# Autodesk Inventor assembly: Spring Assembly
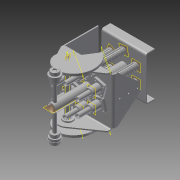
[picture p0: Inventor's stored thumbnail of the model, 180x180]
Saved by Autodesk Inventor 2014 (Build 180170000, 170)
## iProperties
Created: 2014-01-12
Part Number: Spring Assembly
Document SubType Name: Assembly
Designer: Andrew Toennies
Mass: 3782.05 g
Surface Area: 3929.11 cm^2
Volume: 481.789 cm^3
Density: 7.85 g/cm^3
Author: Andrew Toennies
## Documents named in this file (12)
- C:\Users\Andrew Toennies\Documents\GitHub\2014buildCAD\Shooter\Launching Mechanism\Spring Assembly.iam
- C:\Users\Andrew Toennies\Documents\GitHub\2014buildCAD\Shooter\Launching Mechanism\Plate (Front).ipt
- C:\Users\Andrew Toennies\Documents\GitHub\2014buildCAD\Shooter\Launching Mechanism\Spring 9657K213.ipt
- C:\Users\Andrew Toennies\Documents\GitHub\2014buildCAD\Shooter\Launching Mechanism\Shaft (0.500 Aluminum.ipt
- C:\Users\Andrew Toennies\Documents\GitHub\2014buildCAD\Shooter\Launching Mechanism\Plate 2 (Back).ipt
- C:\Users\Andrew Toennies\Documents\GitHub\2014buildCAD\Shooter\Launching Mechanism\Linear Bearing 6483K630.ipt
- C:\Users\Andrew Toennies\Documents\GitHub\2014buildCAD\Shooter\Launching Mechanism\Nautilus Cam.ipt
- C:\Users\Andrew Toennies\Documents\GitHub\2014buildCAD\Shooter\Launching Mechanism\Steel Pipe.ipt
- C:\Users\Andrew Toennies\Documents\GitHub\2014buildCAD\Shooter\Launching Mechanism\Steel Shaft.ipt
- C:\Users\Andrew Toennies\Documents\GitHub\2014buildCAD\Shooter\Launching Mechanism\Steel Shaft 2.ipt
- C:\Users\Andrew Toennies\Documents\GitHub\2014buildCAD\Shooter\Bearing ID 0.500 Hex OD 1.125.ipt
- C:\Users\Andrew Toennies\Documents\GitHub\2014buildCAD\Shooter\Bearing .5 Shaft 6384K610.ipt
## Components (29 placed, 11 different names)
1. Plate (Front):1 — Flush:1, Flush:2, Flush:3, Flush:4, Flush:5, Flush:6, Flush:7, Mate:7, Mate:8, Flush:8, Mate:9, Flush:9, Mate:10, Flush:10, Mate:11, Flush:11, Mate:12, Flush:12, Mate:37, Mate:55, Flush:19
2. Plate 2 (Back):1 — Mate:13, Mate:14, Mate:16, Mate:17, Mate:18, Mate:19, Mate:20, Mate:21, Mate:22, Mate:23, Mate:24, Mate:25, Mate:26, Mate:27, Mate:28, Mate:29, Mate:30, Mate:31, Mate:32, Mate:33, Mate:34, Mate:48, Mate:49, Mate:50, Mate:51, Mate:52, Mate:53, Mate:55
3. Nautilus Cam:1 — Flush:13, Flush:14, Flush:17, Mate:48, Flush:18, Tangent:1
4. Nautilus Cam:2 — Flush:13, Flush:14, Mate:41, Mate:42, Mate:49, Flush:20
5. Steel Pipe:1 — Mate:37, Mate:44, Mate:66, Flush:19
6. Steel Shaft:1 — Mate:41, Mate:42, Flush:17, Mate:54
7. Steel Shaft 2:1 — Mate:44, Mate:64, Mate:65, Mate:66
8. Bearing ID 0.500 Hex OD 1.125:1 — Mate:50, Mate:51, Mate:54
9. Bearing ID 0.500 Hex OD 1.125:2 — Mate:52, Mate:53
10. Bearing .5 Shaft 6384K610:1 — Mate:64, Flush:20
11. Bearing .5 Shaft 6384K610:2 — Mate:65, Flush:18, Tangent:1
12. Spring 9657K213:1 — Flush:5
13. Spring 9657K213:2 — Flush:4
14. Spring 9657K213:3 — Flush:1
15. Spring 9657K213:4 — Flush:2
16. Spring 9657K213:5 — Flush:6
17. Spring 9657K213:6 — Flush:3
18. Shaft (0.500 Aluminum:1 — Mate:11, Flush:11, Mate:14
19. Shaft (0.500 Aluminum:2 — Flush:7, Mate:7
20. Shaft (0.500 Aluminum:3 — Mate:10, Flush:10
21. Shaft (0.500 Aluminum:4 — Mate:12, Flush:12
22. Shaft (0.500 Aluminum:5 — Mate:9, Flush:9, Mate:16
23. Shaft (0.500 Aluminum:6 — Mate:8, Flush:8, Mate:13
24. Linear Bearing 6483K630:1 — Mate:26, Mate:27, Mate:28
25. Linear Bearing 6483K630:2 — Mate:32, Mate:33, Mate:34
26. Linear Bearing 6483K630:3 — Mate:23, Mate:24, Mate:25
27. Linear Bearing 6483K630:4 — Mate:29, Mate:30, Mate:31
28. Linear Bearing 6483K630:5 — Mate:20, Mate:21, Mate:22
29. Linear Bearing 6483K630:6 — Mate:17, Mate:18, Mate:19
## Relationships (61: Mate 42, Flush 18, Tangent 1)
- Flush:1: Plate (Front):1 ↔ Spring 9657K213:3
- Flush:2: Plate (Front):1 ↔ Spring 9657K213:4
- Flush:3: Plate (Front):1 ↔ Spring 9657K213:6
- Flush:4: Plate (Front):1 ↔ Spring 9657K213:2
- Flush:5: Plate (Front):1 ↔ Spring 9657K213:1
- Flush:6: Plate (Front):1 ↔ Spring 9657K213:5
- Flush:7: Plate (Front):1 ↔ Shaft (0.500 Aluminum:2
- Mate:7: Plate (Front):1 ↔ Shaft (0.500 Aluminum:2
- Mate:8: Plate (Front):1 ↔ Shaft (0.500 Aluminum:6
- Flush:8: Plate (Front):1 ↔ Shaft (0.500 Aluminum:6
- Mate:9: Plate (Front):1 ↔ Shaft (0.500 Aluminum:5
- Flush:9: Plate (Front):1 ↔ Shaft (0.500 Aluminum:5
- Mate:10: Plate (Front):1 ↔ Shaft (0.500 Aluminum:3
- Flush:10: Plate (Front):1 ↔ Shaft (0.500 Aluminum:3
- Mate:11: Plate (Front):1 ↔ Shaft (0.500 Aluminum:1
- Flush:11: Plate (Front):1 ↔ Shaft (0.500 Aluminum:1
- Mate:12: Plate (Front):1 ↔ Shaft (0.500 Aluminum:4
- Flush:12: Plate (Front):1 ↔ Shaft (0.500 Aluminum:4
- Mate:13: Plate 2 (Back):1 ↔ Shaft (0.500 Aluminum:6
- Mate:14: Plate 2 (Back):1 ↔ Shaft (0.500 Aluminum:1
- Mate:16: Plate 2 (Back):1 ↔ Shaft (0.500 Aluminum:5
- Mate:17: Plate 2 (Back):1 ↔ Linear Bearing 6483K630:6
- Mate:18: Plate 2 (Back):1 ↔ Linear Bearing 6483K630:6
- Mate:19: Plate 2 (Back):1 ↔ Linear Bearing 6483K630:6
- Mate:20: Plate 2 (Back):1 ↔ Linear Bearing 6483K630:5
- Mate:21: Plate 2 (Back):1 ↔ Linear Bearing 6483K630:5
- Mate:22: Plate 2 (Back):1 ↔ Linear Bearing 6483K630:5
- Mate:23: Plate 2 (Back):1 ↔ Linear Bearing 6483K630:3
- Mate:24: Plate 2 (Back):1 ↔ Linear Bearing 6483K630:3
- Mate:25: Plate 2 (Back):1 ↔ Linear Bearing 6483K630:3
- Mate:26: Plate 2 (Back):1 ↔ Linear Bearing 6483K630:1
- Mate:27: Plate 2 (Back):1 ↔ Linear Bearing 6483K630:1
- Mate:28: Plate 2 (Back):1 ↔ Linear Bearing 6483K630:1
- Mate:29: Plate 2 (Back):1 ↔ Linear Bearing 6483K630:4
- Mate:30: Plate 2 (Back):1 ↔ Linear Bearing 6483K630:4
- Mate:31: Plate 2 (Back):1 ↔ Linear Bearing 6483K630:4
- Mate:32: Plate 2 (Back):1 ↔ Linear Bearing 6483K630:2
- Mate:33: Plate 2 (Back):1 ↔ Linear Bearing 6483K630:2
- Mate:34: Plate 2 (Back):1 ↔ Linear Bearing 6483K630:2
- Flush:13: Nautilus Cam:1 ↔ Nautilus Cam:2
- Flush:14: Nautilus Cam:1 ↔ Nautilus Cam:2
- Mate:37: Plate (Front):1 ↔ Steel Pipe:1
- Mate:41: Nautilus Cam:2 ↔ Steel Shaft:1
- Mate:42: Nautilus Cam:2 ↔ Steel Shaft:1
- Mate:44: Steel Pipe:1 ↔ Steel Shaft 2:1
- Flush:17 (-6.35 mm): Nautilus Cam:1 ↔ Steel Shaft:1
- Mate:48: Plate 2 (Back):1 ↔ Nautilus Cam:1
- Mate:49: Plate 2 (Back):1 ↔ Nautilus Cam:2
- Mate:50: Plate 2 (Back):1 ↔ Bearing ID 0.500 Hex OD 1.125:1
- Mate:51: Plate 2 (Back):1 ↔ Bearing ID 0.500 Hex OD 1.125:1
- Mate:52: Plate 2 (Back):1 ↔ Bearing ID 0.500 Hex OD 1.125:2
- Mate:53: Plate 2 (Back):1 ↔ Bearing ID 0.500 Hex OD 1.125:2
- Mate:54: Steel Shaft:1 ↔ Bearing ID 0.500 Hex OD 1.125:1
- Mate:55: Plate (Front):1 ↔ Plate 2 (Back):1
- Mate:64: Steel Shaft 2:1 ↔ Bearing .5 Shaft 6384K610:1
- Mate:65: Steel Shaft 2:1 ↔ Bearing .5 Shaft 6384K610:2
- Flush:18: Nautilus Cam:1 ↔ Bearing .5 Shaft 6384K610:2
- Mate:66 (-88.9 mm): Steel Pipe:1 ↔ Steel Shaft 2:1
- Flush:19: Plate (Front):1 ↔ Steel Pipe:1
- Tangent:1: Nautilus Cam:1 ↔ Bearing .5 Shaft 6384K610:2
- Flush:20: Nautilus Cam:2 ↔ Bearing .5 Shaft 6384K610:1
